# Autodesk Inventor assembly: UBG-Schusskörper
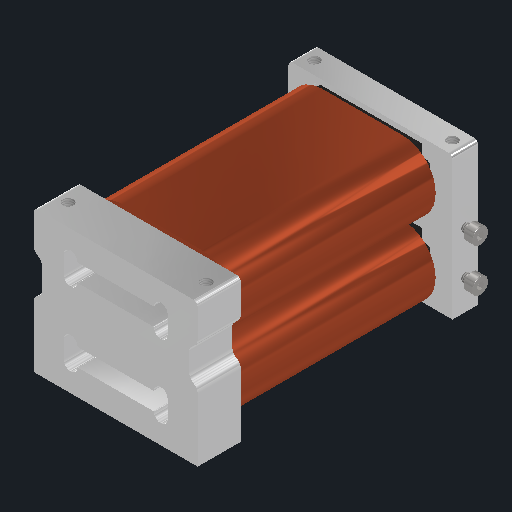
[picture p0: Inventor's stored thumbnail of the model, 512x512]
Saved by Autodesk Inventor 2025.2 (Build 292293000, 293)
## iProperties
Created: 2024-11-08
Part Number: UBG-Schusskörper
Document SubType Name: Assembly
Designer: Fabian
Author: Fabian
## Documents named in this file (5)
- C:\Users\Faabs\Desktop\HBG v2025\Unterbaugruppen\UBG-Schussbauteile\UBG-Schusskörper\UBG-Schusskörper.iam
- C:\Users\Faabs\Desktop\HBG v2025\Unterbaugruppen\UBG-Schussbauteile\UBG-Schusskörper\Bauteile\Spulenhalter Vorne.ipt
- C:\Users\Faabs\Desktop\HBG v2025\Unterbaugruppen\UBG-Schussbauteile\UBG-Spule\UBG-Spule.iam
- C:\Users\Faabs\Desktop\HBG v2025\Unterbaugruppen\UBG-Schussbauteile\UBG-Schusskörper\Bauteile\Spulenhalter Hinten.ipt
- C:\Users\Faabs\Desktop\HBG v2025\Verbindungselemente\DIN 912\DIN 912 - M2 x 0,4 x 6 x 5.ipt
## Components (8 placed, 4 different names)
1. Spulenhalter Vorne:1 — Fluchtend:1, Passend:1, Fluchtend:2, Passend:2, Passend:3, Passend:4, Passend:5, Passend:6, Passend:7, Fluchtend:3, Fluchtend:4
2. UBG-Spule:1 [sub-assembly] — Passend:2, Passend:3, Passend:4, Passend:8
3. UBG-Spule:2 [sub-assembly] — Passend:5, Passend:6, Passend:7
4. Spulenhalter Hinten:1 — Fluchtend:3, Fluchtend:4, Passend:8, Einfügen:1, Einfügen:2, Einfügen:3, Einfügen:4
5. DIN 912 - ersetzt durch DIN EN ISO 4762 M2 x 6:1 — Einfügen:2
6. DIN 912 - ersetzt durch DIN EN ISO 4762 M2 x 6:2 — Einfügen:1
7. DIN 912 - ersetzt durch DIN EN ISO 4762 M2 x 6:3 — Einfügen:4
8. DIN 912 - ersetzt durch DIN EN ISO 4762 M2 x 6:4 — Einfügen:3
## Relationships (16: Mate 8, Flush 4, Insert 4)
- Fluchtend:1 [Flush]: Spulenhalter Vorne:1
- Passend:1 [Mate] (-16.5 mm): Spulenhalter Vorne:1
- Fluchtend:2 [Flush] (-19 mm): Spulenhalter Vorne:1
- Passend:2 [Mate] (0.2 mm): Spulenhalter Vorne:1 ↔ UBG-Spule:1
- Passend:3 [Mate] (0.2 mm): Spulenhalter Vorne:1 ↔ UBG-Spule:1
- Passend:4 [Mate] (0.1 mm): Spulenhalter Vorne:1 ↔ UBG-Spule:1
- Passend:5 [Mate] (0.2 mm): Spulenhalter Vorne:1 ↔ UBG-Spule:2
- Passend:6 [Mate] (0.2 mm): Spulenhalter Vorne:1 ↔ UBG-Spule:2
- Passend:7 [Mate] (0.1 mm): Spulenhalter Vorne:1 ↔ UBG-Spule:2
- Fluchtend:3 [Flush]: Spulenhalter Vorne:1 ↔ Spulenhalter Hinten:1
- Fluchtend:4 [Flush]: Spulenhalter Vorne:1 ↔ Spulenhalter Hinten:1
- Passend:8 [Mate] (0.1 mm): UBG-Spule:1 ↔ Spulenhalter Hinten:1
- Einfügen:1 [Insert] (1.5 mm): Spulenhalter Hinten:1 ↔ DIN 912 - ersetzt durch DIN EN ISO 4762 M2 x 6:2
- Einfügen:2 [Insert] (1.5 mm): Spulenhalter Hinten:1 ↔ DIN 912 - ersetzt durch DIN EN ISO 4762 M2 x 6:1
- Einfügen:3 [Insert] (1.5 mm): Spulenhalter Hinten:1 ↔ DIN 912 - ersetzt durch DIN EN ISO 4762 M2 x 6:4
- Einfügen:4 [Insert] (1.5 mm): Spulenhalter Hinten:1 ↔ DIN 912 - ersetzt durch DIN EN ISO 4762 M2 x 6:3
